# Autodesk Inventor assembly: Assembly_base_4x1
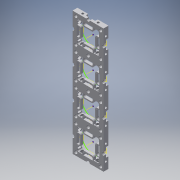
[picture p0: Inventor's stored thumbnail of the model, 180x180]
Saved by Autodesk Inventor 2019 (Build 230136000, 136)
## iProperties
Created: 2018-11-29
Part Number: Assembly_base_4x1
Document SubType Name: Assembly
Designer: marsikovabarbora
Author: marsikovabarbora
## Documents named in this file (2)
- C:\Users\marsikovabarbora.IPHT-JENA\Documents\Inventor\cube\Assembly_base_4x1.iam
- U:\Inventor\10_Cube_Base\Assembly_base_1x2.iam
## Components (2 placed, 1 different names)
1. Assembly_base_1x2:1 [sub-assembly] — Mate:1, Mate:2
2. Assembly_base_1x2:2 [sub-assembly] — Mate:1, Mate:2
## Relationships (2: Mate 2)
- Mate:1: Assembly_base_1x2:1 ↔ Assembly_base_1x2:2
- Mate:2: Assembly_base_1x2:1 ↔ Assembly_base_1x2:2
